# Autodesk Inventor assembly: Spinning Platform
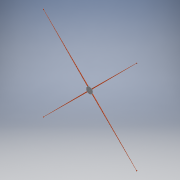
[picture p0: Inventor's stored thumbnail of the model, 180x180]
Saved by Autodesk Inventor 2016 (Build 200138000, 138)
## iProperties
Created: 2016-01-01
Part Number: Spinning Platform
Document SubType Name: Assembly
Designer: jonathan
Author: jonathan
## Documents named in this file (3)
- C:\Users\jonathan\Dropbox\Satellite\CAD\Spinning Platform.iam
- C:\Users\jonathan\Dropbox\Satellite\CAD\Boom Platform.ipt
- C:\Users\jonathan\Dropbox\Satellite\CAD\STACER.ipt
## Components (5 placed, 2 different names)
1. Boom Platform:1 — Flush:1, Mate:1, Flush:2, Mate:2, Flush:3, Mate:3, Flush:4, Mate:4
2. STACER:1 — Flush:1, Mate:1
3. STACER:2 — Flush:2, Mate:2
4. STACER:3 — Flush:3, Mate:3
5. STACER:4 — Flush:4, Mate:4
## Relationships (8: Flush 4, Mate 4)
- Flush:1: Boom Platform:1 ↔ STACER:1
- Mate:1: Boom Platform:1 ↔ STACER:1
- Flush:2: Boom Platform:1 ↔ STACER:2
- Mate:2: Boom Platform:1 ↔ STACER:2
- Flush:3: Boom Platform:1 ↔ STACER:3
- Mate:3: Boom Platform:1 ↔ STACER:3
- Flush:4: Boom Platform:1 ↔ STACER:4
- Mate:4: Boom Platform:1 ↔ STACER:4
